# Autodesk Inventor assembly: xy-motion-asm
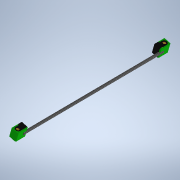
[picture p0: Inventor's stored thumbnail of the model, 180x180]
Saved by Autodesk Inventor 2020.4 (Build 244396000, 396)
## iProperties
Created: 2021-03-31
Part Number: xy-motion-asm
Document SubType Name: Assembly
Designer: AOB
Mass: 84.8911 g
Surface Area: 402.633 cm^2
Volume: 35.3413 cm^3
Density: 2.40203 g/cm^3
Author: AOB
## Documents named in this file (3)
- C:\Users\marti\Documents\Inventor\ProjectBoron\Boron Ultima\xy-motion-asm.iam
- C:\Users\marti\Documents\Inventor\ProjectBoron\Boron Ultima\Y-linear bearing shroud.iam
- C:\Users\marti\Documents\Inventor\ProjectBoron\Boron Ultima\8mm carbon fiber rod.ipt
## Components (3 placed, 2 different names)
1. Y-linear bearing shroud:1 [sub-assembly] — Rigid:3
2. Y-linear bearing shroud:2 [sub-assembly] — Rigid:4
3. 8mm carbon fiber rod:2 — Rigid:3, Rigid:4
## Relationships (2: WeldJoint 2)
- Rigid:3 [WeldJoint] (-9.5399 mm): Y-linear bearing shroud:1 ↔ 8mm carbon fiber rod:2
- Rigid:4 [WeldJoint] (9.5399 mm): Y-linear bearing shroud:2 ↔ 8mm carbon fiber rod:2
